# Autodesk Inventor assembly: ASM Frame
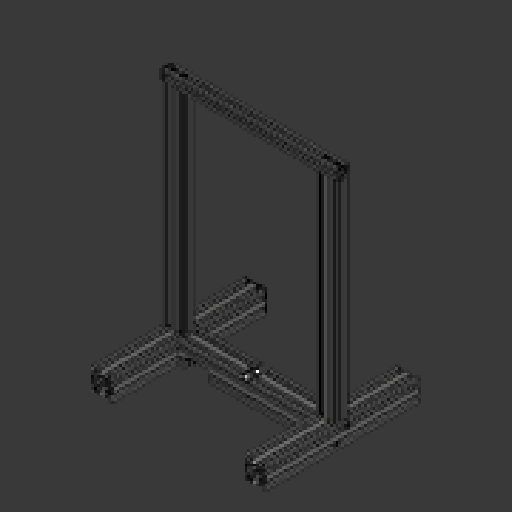
[picture p0: Inventor's stored thumbnail of the model, 512x512]
Saved by Autodesk Inventor 2023 (Build 270158000, 158)
## iProperties
Created: 2018-08-16
Part Number: ASM Frame
Document SubType Name: Assembly
Designer: alber
Sending System: SolidWorks 2015
Last Author: Poseidon
Last Saved: 2018-08-17
Author: alber
## Documents named in this file (10)
- C:\Users\alber\Desktop\Files\Ender3-Upgrade\CAD\ASM Frame.iam
- C:\Users\alber\Desktop\Files\Ender3-Upgrade\CAD\4040 profile.ipt
- C:\Users\alber\Desktop\Files\Ender3-Upgrade\CAD\4040-3 profile.ipt
- C:\Users\alber\Desktop\Files\Ender3-Upgrade\CAD\2020-2 profile.ipt
- C:\Users\alber\Desktop\Files\Ender3-Upgrade\CAD\2040-3R profile.ipt
- C:\Users\alber\Desktop\Files\Ender3-Upgrade\CAD\2040-3L profile.ipt
- C:\Users\alber\Desktop\Files\Ender3-Upgrade\CAD\2020 Endcap.ipt
- C:\Users\alber\Desktop\Files\Ender3-Upgrade\CAD\M5X45 Socket Head Screw.ipt
- C:\Users\alber\Desktop\Files\Ender3-Upgrade\CAD\LED Holder.ipt
- C:\Users\alber\Desktop\Files\Ender3-Upgrade\CAD\LED Holder Magnetic.ipt
## Components (27 placed, 9 different names)
1. 4040 profile:1
2. 4040 profile:2
3. 4040-3 profile:1
4. 2020-2 profile:1 — Mate:1, Mate:2
5. 2040-3R profile:1
6. 2040-3L profile:1
7. 2020 Endcap:1
8. 2020 Endcap:2
9. 2020 Endcap:4
10. M5X45 Socket Head Screw:1
11. M5X45 Socket Head Screw:2
12. M5X45 Socket Head Screw:3
13. M5X45 Socket Head Screw:4
14. M5X45 Socket Head Screw:5
15. M5X45 Socket Head Screw:6
16. M5X45 Socket Head Screw:7
17. M5X45 Socket Head Screw:8
18. M5X45 Socket Head Screw:9
19. M5X45 Socket Head Screw:10
20. M5X45 Socket Head Screw:12
21. M5X45 Socket Head Screw:13
22. M5X45 Socket Head Screw:14
23. 2020 Endcap:5
24. 2020 Endcap:6
25. 2020 Endcap:7
26. LED Holder:1 — Mate:1, Mate:2, Flush:1, Flush:2
27. LED Holder Magnetic:1 — Flush:1, Flush:2
## Relationships (4: Mate 2, Flush 2)
- Mate:1: 2020-2 profile:1 ↔ LED Holder:1
- Mate:2 (0.5 mm): 2020-2 profile:1 ↔ LED Holder:1
- Flush:1: LED Holder:1 ↔ LED Holder Magnetic:1
- Flush:2: LED Holder:1 ↔ LED Holder Magnetic:1
